# Autodesk Inventor assembly: 200-02-ROCKER-CONNECTOR-ASM-L
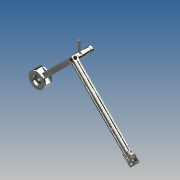
[picture p0: Inventor's stored thumbnail of the model, 180x180]
Saved by Autodesk Inventor 2018.2 (Build 222227000, 227)
## iProperties
Manager: feesmrt
Company: FRANC0R
Created: 2017-12-19
Part Number: 200-02-ROCKER-CONNECTOR-ASM-L
Project: Rescue Robot
Cost Center: -
Material: Generisch
Document SubType Name: Assembly
Designer: feesmrt
Engineer: feesmrt
Authority: feesmrt
Description: Rocker Connector Left Side ASM
Stock Number: 200-02-ROCKER-CONNECTOR-ASM-L
Subject: Rescue Robot
Author: feesmrt
Revision Number: 1
Title: Rocker Connector Left Side ASM
## Documents named in this file (6)
- D:\Programmierung\FRANC0R\CAD\02-Rocker-Bogie-Robot\200-ROCKER-BOGIE\200-02-ROCKER-CONNECTOR-ASM-L.iam
- D:\Programmierung\FRANC0R\CAD\02-Rocker-Bogie-Robot\200-ROCKER-BOGIE\200-20-ROCKER-CONNECTOR\200-20-ROCKER-CONNECTOR-ASM-01.iam
- D:\Programmierung\FRANC0R\CAD\02-Rocker-Bogie-Robot\900-COMPONENTS\900-50-PROFILES\90-50-PROFILES-30x30x250.ipt
- D:\Programmierung\FRANC0R\CAD\02-Rocker-Bogie-Robot\900-COMPONENTS\900-50-PROFILES\90-50-PROFILES-30x30x500.ipt
- D:\Programmierung\FRANC0R\CAD\02-Rocker-Bogie-Robot\200-ROCKER-BOGIE\200-30-BOGIE-BEARING\200-30-BOGIE-BEARING-ASM-01.iam
- D:\Programmierung\FRANC0R\CAD\02-Rocker-Bogie-Robot\200-ROCKER-BOGIE\200-50-WHEEL-CONNECTOR\200-50-WHEEL-CONNECTOR-30MM-ASM-01.iam
## Components (5 placed, 5 different names)
1. 200-20-ROCKER-CONNECTOR-ASM-01:1 [sub-assembly] — Passend:1, Passend:2, Winkel:1, Passend:3, Passend:4, Winkel:2
2. 90-50-PROFILES-30x30x250:1 — Passend:3, Passend:4, Winkel:2, Passend:5, Passend:6, Fluchtend:1
3. 90-50-PROFILES-30x30x500:1 — Passend:1, Passend:2, Winkel:1, Passend:7, Fluchtend:2, Passend:8
4. 200-30-BOGIE-BEARING-ASM-01:1 [sub-assembly] — Passend:5, Passend:6, Fluchtend:1
5. 200-50-WHEEL-CONNECTOR-30MM-ASM-01:1 [sub-assembly] — Passend:7, Fluchtend:2, Passend:8
## Relationships (12: Mate 8, Angle 2, Flush 2)
- Passend:1 [Mate]: 200-20-ROCKER-CONNECTOR-ASM-01:1 ↔ 90-50-PROFILES-30x30x500:1
- Passend:2 [Mate]: 200-20-ROCKER-CONNECTOR-ASM-01:1 ↔ 90-50-PROFILES-30x30x500:1
- Winkel:1 [Angle] (0 deg): 200-20-ROCKER-CONNECTOR-ASM-01:1 ↔ 90-50-PROFILES-30x30x500:1
- Passend:3 [Mate]: 200-20-ROCKER-CONNECTOR-ASM-01:1 ↔ 90-50-PROFILES-30x30x250:1
- Passend:4 [Mate]: 200-20-ROCKER-CONNECTOR-ASM-01:1 ↔ 90-50-PROFILES-30x30x250:1
- Winkel:2 [Angle] (0 deg): 200-20-ROCKER-CONNECTOR-ASM-01:1 ↔ 90-50-PROFILES-30x30x250:1
- Passend:5 [Mate]: 90-50-PROFILES-30x30x250:1 ↔ 200-30-BOGIE-BEARING-ASM-01:1
- Passend:6 [Mate]: 90-50-PROFILES-30x30x250:1 ↔ 200-30-BOGIE-BEARING-ASM-01:1
- Fluchtend:1 [Flush]: 90-50-PROFILES-30x30x250:1 ↔ 200-30-BOGIE-BEARING-ASM-01:1
- Passend:7 [Mate]: 90-50-PROFILES-30x30x500:1 ↔ 200-50-WHEEL-CONNECTOR-30MM-ASM-01:1
- Fluchtend:2 [Flush]: 90-50-PROFILES-30x30x500:1 ↔ 200-50-WHEEL-CONNECTOR-30MM-ASM-01:1
- Passend:8 [Mate]: 90-50-PROFILES-30x30x500:1 ↔ 200-50-WHEEL-CONNECTOR-30MM-ASM-01:1
